# Autodesk Inventor assembly: RearLeg
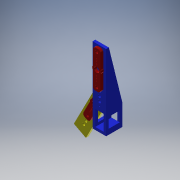
[picture p0: Inventor's stored thumbnail of the model, 180x180]
Saved by Autodesk Inventor 2019 (Build 230136000, 136)
## iProperties
Created: 2019-04-01
Part Number: RearLeg
Document SubType Name: Assembly
Designer: cnam
Author: cnam
## Documents named in this file (4)
- \\engrfs904v\VCL.userspace\cnam\Documents\RearLeg.iam
- \\engrfs904v\VCL.userspace\cnam\Documents\BottomRearLeg.ipt
- \\engrfs904v\VCL.userspace\cnam\Documents\TopRearLeg.ipt
- \\engrfs904v\VCL.userspace\cnam\Documents\JointPlate.ipt
## Components (4 placed, 3 different names)
1. BottomRearLeg:1 — Mate:3, Mate:4, Mate:5
2. TopRearLeg:1 — Rotational:1, Mate:1, Mate:2
3. JointPlate:1 — Rotational:1, Mate:1
4. JointPlate:2 — Mate:2, Mate:3, Mate:4, Mate:5
## Relationships (6: Mate 5, RevoluteJoint 1)
- Rotational:1 [RevoluteJoint]: TopRearLeg:1 ↔ JointPlate:1
- Mate:1: TopRearLeg:1 ↔ JointPlate:1
- Mate:2: TopRearLeg:1 ↔ JointPlate:2
- Mate:3: BottomRearLeg:1 ↔ JointPlate:2
- Mate:4: BottomRearLeg:1 ↔ JointPlate:2
- Mate:5: BottomRearLeg:1 ↔ JointPlate:2
